# Autodesk Inventor assembly: zlozenie
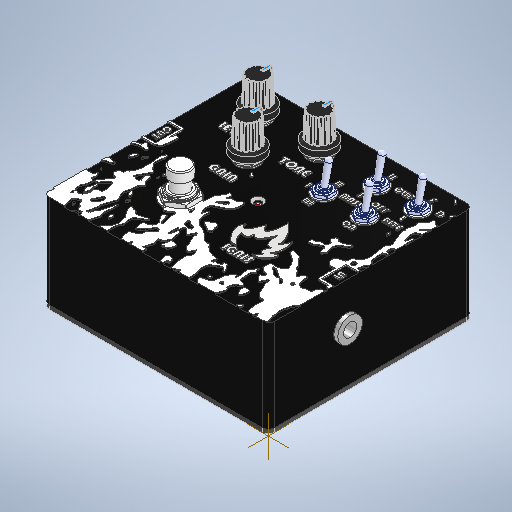
[picture p0: Inventor's stored thumbnail of the model, 512x512]
Saved by Autodesk Inventor 2025 (Build 290162000, 162)
## iProperties
Created: 2026-04-02
Part Number: zlozenie
Document SubType Name: Assembly
Designer: zzapa
Author: zzapa
## Documents named in this file (18)
- C:\Users\zzapa\Desktop\Projekty\elektronika\Ignis-overdrive\model\assembly.iam
- C:\Users\zzapa\Desktop\Projekty\elektronika\Ignis-overdrive\model\base.ipt
- C:\Users\zzapa\Desktop\Projekty\elektronika\Ignis-overdrive\model\enclosure.ipt
- C:\Users\zzapa\Documents\Inventor\Content Center Files\R2025\pl-PL\GB 809-88 B\Nut GB 809 B M2,5 x 6.ipt
- C:\Users\zzapa\Desktop\Projekty\elektronika\Ignis-overdrive\model\PotentiometerB10K.ipt
- C:\Users\zzapa\Desktop\Projekty\elektronika\Ignis-overdrive\model\knob.ipt
- C:\Users\zzapa\Desktop\Projekty\elektronika\Ignis-overdrive\model\Jack_enclosure.ipt
- C:\Users\zzapa\Desktop\Projekty\elektronika\Ignis-overdrive\model\Jack_inner.ipt
- C:\Users\zzapa\Desktop\Projekty\elektronika\Ignis-overdrive\model\9V_battery.ipt
- C:\Users\zzapa\Desktop\Projekty\elektronika\Ignis-overdrive\model\9V_input.ipt
- C:\Users\zzapa\Desktop\Projekty\elektronika\Ignis-overdrive\model\import\MTS-1xx-A1-blue\MTS-1xx-A1-blue-no-nuts.iam
- C:\Users\zzapa\Desktop\Projekty\elektronika\Ignis-overdrive\model\import\PCB_V1\PCB_V1.iam
- C:\Users\zzapa\Desktop\Projekty\elektronika\Ignis-overdrive\model\import\GŘRVA_MECHANO_3PDT_FOOTSWITCH\GŘRVA_MECHANO_3PDT_FOOTSWITCH.ipt
- C:\Users\zzapa\Desktop\Projekty\elektronika\Ignis-overdrive\model\import\M7 × 0.75 NUT\M7 × 0.75 NUT.ipt
- C:\Users\zzapa\Desktop\Projekty\elektronika\Ignis-overdrive\model\import\M12 NUT FOR FOOTSWITCH\M12 NUT FOR FOOTSWITCH.ipt
- C:\Users\zzapa\Desktop\Projekty\elektronika\Ignis-overdrive\model\import\MTS-1xx-A1-blue\MTS-1xx-NUT.ipt
- C:\Users\zzapa\Desktop\Projekty\elektronika\Ignis-overdrive\model\import\red-led-5mm\red-led-5mm.ipt
- C:\Users\zzapa\Desktop\Projekty\elektronika\Ignis-overdrive\model\led_holder.ipt
## Components (40 placed, 17 different names)
1. base:1 — Zestawiające:1, Zestawiające:2, Zestawiające:3, Zestawiające:4, Zestawiające:9, Zestawiające:87, Równoległe:19, Zestawiające:88
2. enclosure:1 — Zestawiające:3, Zestawiające:4, Zestawiające:5, Równoległe:1, Zestawiające:6, Równoległe:2, Zestawiające:7, Równoległe:3, Zestawiające:8, Równoległe:4, Zestawiające:9, Zestawiające:23, Zestawiające:24, Zestawiające:25, Zestawiające:26, Zestawiające:27, Zestawiające:28, Zestawiające:29, Równoległe:5, Zestawiające:32, Zestawiające:33, Zestawiające:47, Zestawiające:48, Zestawiające:49, Zestawiające:50, Zestawiające:51, Zestawiające:52, Zestawiające:53, Równoległe:10, Równoległe:11, Równoległe:12, Równoległe:13, Zestawiające:63, Zestawiające:64, Zestawiające:65, Zestawiające:66, Zestawiające:67, Zestawiające:68, Zestawiające:72, Zestawiające:74, Zestawiające:75, Zestawiające:76, Zestawiające:77, Zestawiające:78, Zestawiające:83, Zestawiające:84, Zestawiające:85, Zestawiające:86, Kątowe:43, Zestawiające:89, Zestawiające:90, Zestawiające:93, Zestawiające:94, Zestawiające:95, Równoległe:20, Równoległe:21
3. Nut GB/T 809-1988 Type B M2,5x6:1 — Zestawiające:5, Równoległe:1, Kątowe:1
4. Nut GB/T 809-1988 Type B M2,5x6:2 — Zestawiające:6, Równoległe:2, Kątowe:2
5. Nut GB/T 809-1988 Type B M2,5x6:3 — Zestawiające:7, Równoległe:3, Kątowe:3
6. Nut GB/T 809-1988 Type B M2,5x6:4 — Zestawiające:8, Równoległe:4, Kątowe:4
7. PotentiometerB10K:1 — Kątowe:5, Zestawiające:18, Zestawiające:19, Zestawiające:54
8. PotentiometerB10K:2 — Kątowe:6, Zestawiające:17, Zestawiające:20, Zestawiające:57
9. PotentiometerB10K:3 — Kątowe:7, Zestawiające:16, Zestawiające:21, Zestawiające:56
10. knob:1 — Zestawiające:17, Zestawiające:20, Kątowe:12, Zestawiające:71
11. knob:2 — Zestawiające:16, Zestawiające:21, Kątowe:13, Zestawiające:70
12. knob:3 — Zestawiające:18, Zestawiające:19, Kątowe:14, Zestawiające:69
13. Jack_enclosure:1 — Zestawiające:22, Zestawiające:25, Kątowe:11
14. Jack_inner:1 — Zestawiające:22, Zestawiające:23, Zestawiające:24, Kątowe:10
15. Jack_enclosure:2 — Zestawiające:26, Zestawiające:27, Kątowe:9
16. Jack_inner:2 — Zestawiające:28, Zestawiające:29, Kątowe:8
17. 9V_battery:1 — Kątowe:43, Zestawiające:87, Równoległe:19, Zestawiające:88
18. 9V_input:1 — Równoległe:5, Zestawiające:32, Zestawiające:33
19. PCB_V1:1 [sub-assembly] — Zestawiające:47, Zestawiające:48, Zestawiające:49
20. GŘRVA_MECHANO_3PDT_FOOTSWITCH:1 — Zestawiające:72, Zestawiające:73, Równoległe:14, Kątowe:34
21. Nut GB/T 809-1988 Type B M2,5x6:5 — Zestawiające:50, Równoległe:12, Kątowe:26
22. Nut GB/T 809-1988 Type B M2,5x6:6 — Zestawiające:52, Równoległe:11, Kątowe:27
23. Nut GB/T 809-1988 Type B M2,5x6:7 — Zestawiające:53, Równoległe:10, Kątowe:28
24. Nut GB/T 809-1988 Type B M2,5x6:8 — Zestawiające:51, Równoległe:13, Kątowe:29
25. M7 × 0.75 NUT:1 — Zestawiające:54, Kątowe:30, Zestawiające:66, Zestawiające:67, Zestawiające:69
26. M7 × 0.75 NUT:2 — Zestawiające:56, Kątowe:31, Zestawiające:63, Zestawiające:68, Zestawiające:70
27. M7 × 0.75 NUT:3 — Kątowe:32, Zestawiające:57, Zestawiające:64, Zestawiające:65, Zestawiające:71
28. M12 NUT FOR FOOTSWITCH:1 — Kątowe:33, Zestawiające:73, Równoległe:14, Zestawiające:74
29. MTS-1xx-A1-blue-no-nuts:1 [sub-assembly] — Zestawiające:75, Zestawiające:80, Równoległe:16, Kątowe:39
30. MTS-1xx-A1-blue-no-nuts:2 [sub-assembly] — Zestawiające:76, Zestawiające:81, Równoległe:18, Kątowe:40
31. MTS-1xx-A1-blue-no-nuts:3 [sub-assembly] — Zestawiające:77, Zestawiające:79, Równoległe:15, Kątowe:41
32. MTS-1xx-A1-blue-no-nuts:4 [sub-assembly] — Zestawiające:78, Zestawiające:82, Równoległe:17, Kątowe:42
33. MTS-1xx-NUT:1 — Zestawiające:82, Kątowe:35, Zestawiające:84, Równoległe:17
34. MTS-1xx-NUT:2 — Zestawiające:81, Kątowe:36, Zestawiające:83, Równoległe:18
35. MTS-1xx-NUT:3 — Zestawiające:80, Kątowe:37, Zestawiające:85, Równoległe:16
36. MTS-1xx-NUT:4 — Zestawiające:79, Kątowe:38, Zestawiające:86, Równoległe:15
37. red-led-5mm:1 — Zestawiające:91, Zestawiające:92, Zestawiające:93
38. led_holder:1 — Zestawiające:89, Zestawiające:90, Zestawiające:91, Zestawiające:92
39. Nut GB/T 809-1988 Type B M2,5x6:9 — Zestawiające:95, Równoległe:21
40. Nut GB/T 809-1988 Type B M2,5x6:10 — Zestawiające:94, Równoległe:20
## Relationships (117: Mate 68, Angle 32, Flush 17)
- Zestawiające:1 [Mate]: base:1
- Zestawiające:2 [Mate]: base:1
- Zestawiające:3 [Mate]: base:1 ↔ enclosure:1
- Zestawiające:4 [Mate]: base:1 ↔ enclosure:1
- Zestawiające:5 [Mate]: enclosure:1 ↔ Nut GB/T 809-1988 Type B M2,5x6:1
- Równoległe:1 [Flush]: enclosure:1 ↔ Nut GB/T 809-1988 Type B M2,5x6:1
- Zestawiające:6 [Mate]: enclosure:1 ↔ Nut GB/T 809-1988 Type B M2,5x6:2
- Równoległe:2 [Flush]: enclosure:1 ↔ Nut GB/T 809-1988 Type B M2,5x6:2
- Zestawiające:7 [Mate]: enclosure:1 ↔ Nut GB/T 809-1988 Type B M2,5x6:3
- Równoległe:3 [Flush]: enclosure:1 ↔ Nut GB/T 809-1988 Type B M2,5x6:3
- Zestawiające:8 [Mate]: enclosure:1 ↔ Nut GB/T 809-1988 Type B M2,5x6:4
- Równoległe:4 [Flush]: enclosure:1 ↔ Nut GB/T 809-1988 Type B M2,5x6:4
- Kątowe:1 [Angle] (0 deg): Nut GB/T 809-1988 Type B M2,5x6:1
- Kątowe:2 [Angle] (0 deg): Nut GB/T 809-1988 Type B M2,5x6:2
- Kątowe:3 [Angle] (0 deg): Nut GB/T 809-1988 Type B M2,5x6:3
- Kątowe:4 [Angle] (0 deg): Nut GB/T 809-1988 Type B M2,5x6:4
- Zestawiające:9 [Mate]: base:1 ↔ enclosure:1
- Kątowe:5 [Angle] (0 deg): PotentiometerB10K:1
- Kątowe:6 [Angle] (0 deg): PotentiometerB10K:2
- Kątowe:7 [Angle] (0 deg): PotentiometerB10K:3
- Zestawiające:16 [Mate]: PotentiometerB10K:3 ↔ knob:2
- Zestawiające:17 [Mate]: PotentiometerB10K:2 ↔ knob:1
- Zestawiające:18 [Mate]: PotentiometerB10K:1 ↔ knob:3
- Zestawiające:19 [Mate]: PotentiometerB10K:1 ↔ knob:3
- Zestawiające:20 [Mate]: PotentiometerB10K:2 ↔ knob:1
- Zestawiające:21 [Mate]: PotentiometerB10K:3 ↔ knob:2
- Zestawiające:22 [Mate]: Jack_enclosure:1 ↔ Jack_inner:1
- Zestawiające:23 [Mate]: enclosure:1 ↔ Jack_inner:1
- Zestawiające:24 [Mate]: enclosure:1 ↔ Jack_inner:1
- Zestawiające:25 [Mate]: enclosure:1 ↔ Jack_enclosure:1
- Zestawiające:26 [Mate]: enclosure:1 ↔ Jack_enclosure:2
- Zestawiające:27 [Mate]: enclosure:1 ↔ Jack_enclosure:2
- Zestawiające:28 [Mate]: enclosure:1 ↔ Jack_inner:2
- Zestawiające:29 [Mate]: enclosure:1 ↔ Jack_inner:2
- Kątowe:8 [Angle] (0 deg): Jack_inner:2
- Kątowe:9 [Angle] (0 deg): Jack_enclosure:2
- Kątowe:10 [Angle] (0 deg): Jack_inner:1
- Kątowe:11 [Angle] (0 deg): Jack_enclosure:1
- Równoległe:5 [Flush]: enclosure:1 ↔ 9V_input:1
- Zestawiające:32 [Mate]: enclosure:1 ↔ 9V_input:1
- Zestawiające:33 [Mate]: enclosure:1 ↔ 9V_input:1
- Kątowe:12 [Angle] (180 deg): knob:1
- Kątowe:13 [Angle] (180 deg): knob:2
- Kątowe:14 [Angle] (180 deg): knob:3
- Zestawiające:47 [Mate]: enclosure:1 ↔ PCB_V1:1
- Zestawiające:48 [Mate]: enclosure:1 ↔ PCB_V1:1
- Zestawiające:49 [Mate]: enclosure:1 ↔ PCB_V1:1
- Zestawiające:50 [Mate]: enclosure:1 ↔ Nut GB/T 809-1988 Type B M2,5x6:5
- Zestawiające:51 [Mate]: enclosure:1 ↔ Nut GB/T 809-1988 Type B M2,5x6:8
- Zestawiające:52 [Mate]: enclosure:1 ↔ Nut GB/T 809-1988 Type B M2,5x6:6
- Zestawiające:53 [Mate]: enclosure:1 ↔ Nut GB/T 809-1988 Type B M2,5x6:7
- Równoległe:10 [Flush]: enclosure:1 ↔ Nut GB/T 809-1988 Type B M2,5x6:7
- Równoległe:11 [Flush]: enclosure:1 ↔ Nut GB/T 809-1988 Type B M2,5x6:6
- Równoległe:12 [Flush]: enclosure:1 ↔ Nut GB/T 809-1988 Type B M2,5x6:5
- Równoległe:13 [Flush]: enclosure:1 ↔ Nut GB/T 809-1988 Type B M2,5x6:8
- Kątowe:26 [Angle] (0 deg): Nut GB/T 809-1988 Type B M2,5x6:5
- Kątowe:27 [Angle] (0 deg): Nut GB/T 809-1988 Type B M2,5x6:6
- Kątowe:28 [Angle] (0 deg): Nut GB/T 809-1988 Type B M2,5x6:7
- Kątowe:29 [Angle] (0 deg): Nut GB/T 809-1988 Type B M2,5x6:8
- Zestawiające:54 [Mate]: PotentiometerB10K:1 ↔ M7 × 0.75 NUT:1
- Zestawiające:56 [Mate]: PotentiometerB10K:3 ↔ M7 × 0.75 NUT:2
- Kątowe:30 [Angle] (0 deg): M7 × 0.75 NUT:1
- Kątowe:31 [Angle] (0 deg): M7 × 0.75 NUT:2
- Kątowe:32 [Angle] (0 deg): M7 × 0.75 NUT:3
- Zestawiające:57 [Mate]: PotentiometerB10K:2 ↔ M7 × 0.75 NUT:3
- Kątowe:33 [Angle] (0 deg): M12 NUT FOR FOOTSWITCH:1
- Zestawiające:63 [Mate]: enclosure:1 ↔ M7 × 0.75 NUT:2
- Zestawiające:64 [Mate]: enclosure:1 ↔ M7 × 0.75 NUT:3
- Zestawiające:65 [Mate]: enclosure:1 ↔ M7 × 0.75 NUT:3
- Zestawiające:66 [Mate]: enclosure:1 ↔ M7 × 0.75 NUT:1
- Zestawiające:67 [Mate]: enclosure:1 ↔ M7 × 0.75 NUT:1
- Zestawiające:68 [Mate]: enclosure:1 ↔ M7 × 0.75 NUT:2
- Zestawiające:69 [Mate] (1 mm): knob:3 ↔ M7 × 0.75 NUT:1
- Zestawiające:70 [Mate] (1 mm): knob:2 ↔ M7 × 0.75 NUT:2
- Zestawiające:71 [Mate] (1 mm): knob:1 ↔ M7 × 0.75 NUT:3
- Zestawiające:72 [Mate]: enclosure:1 ↔ GŘRVA_MECHANO_3PDT_FOOTSWITCH:1
- Zestawiające:73 [Mate]: GŘRVA_MECHANO_3PDT_FOOTSWITCH:1 ↔ M12 NUT FOR FOOTSWITCH:1
- Równoległe:14 [Flush] (1.5 mm): GŘRVA_MECHANO_3PDT_FOOTSWITCH:1 ↔ M12 NUT FOR FOOTSWITCH:1
- Zestawiające:74 [Mate]: enclosure:1 ↔ M12 NUT FOR FOOTSWITCH:1
- Kątowe:34 [Angle] (0 deg): GŘRVA_MECHANO_3PDT_FOOTSWITCH:1
- Zestawiające:75 [Mate]: enclosure:1 ↔ MTS-1xx-A1-blue-no-nuts:1
- Zestawiające:76 [Mate]: enclosure:1 ↔ MTS-1xx-A1-blue-no-nuts:2
- Zestawiające:77 [Mate]: enclosure:1 ↔ MTS-1xx-A1-blue-no-nuts:3
- Zestawiające:78 [Mate]: enclosure:1 ↔ MTS-1xx-A1-blue-no-nuts:4
- Zestawiające:79 [Mate]: MTS-1xx-A1-blue-no-nuts:3 ↔ MTS-1xx-NUT:4
- Zestawiające:80 [Mate]: MTS-1xx-A1-blue-no-nuts:1 ↔ MTS-1xx-NUT:3
- Zestawiające:81 [Mate]: MTS-1xx-A1-blue-no-nuts:2 ↔ MTS-1xx-NUT:2
- Zestawiające:82 [Mate]: MTS-1xx-A1-blue-no-nuts:4 ↔ MTS-1xx-NUT:1
- Kątowe:35 [Angle] (0 deg): MTS-1xx-NUT:1
- Kątowe:36 [Angle] (0 deg): MTS-1xx-NUT:2
- Kątowe:37 [Angle] (0 deg): MTS-1xx-NUT:3
- Kątowe:38 [Angle] (0 deg): MTS-1xx-NUT:4
- Zestawiające:83 [Mate]: enclosure:1 ↔ MTS-1xx-NUT:2
- Zestawiające:84 [Mate]: enclosure:1 ↔ MTS-1xx-NUT:1
- Zestawiające:85 [Mate]: enclosure:1 ↔ MTS-1xx-NUT:3
- Zestawiające:86 [Mate]: enclosure:1 ↔ MTS-1xx-NUT:4
- Równoległe:15 [Flush] (-1 mm): MTS-1xx-A1-blue-no-nuts:3 ↔ MTS-1xx-NUT:4
- Równoległe:16 [Flush] (-1 mm): MTS-1xx-A1-blue-no-nuts:1 ↔ MTS-1xx-NUT:3
- Równoległe:17 [Flush] (-1 mm): MTS-1xx-A1-blue-no-nuts:4 ↔ MTS-1xx-NUT:1
- Równoległe:18 [Flush] (-1 mm): MTS-1xx-A1-blue-no-nuts:2 ↔ MTS-1xx-NUT:2
- Kątowe:39 [Angle] (0 deg): MTS-1xx-A1-blue-no-nuts:1
- Kątowe:40 [Angle] (0 deg): MTS-1xx-A1-blue-no-nuts:2
- Kątowe:41 [Angle] (0 deg): MTS-1xx-A1-blue-no-nuts:3
- Kątowe:42 [Angle] (0 deg): MTS-1xx-A1-blue-no-nuts:4
- Kątowe:43 [Angle] (0 deg): enclosure:1 ↔ 9V_battery:1
- Zestawiające:87 [Mate]: base:1 ↔ 9V_battery:1
- Równoległe:19 [Flush]: base:1 ↔ 9V_battery:1
- Zestawiające:88 [Mate]: base:1 ↔ 9V_battery:1
- Zestawiające:89 [Mate]: enclosure:1 ↔ led_holder:1
- Zestawiające:90 [Mate]: enclosure:1 ↔ led_holder:1
- Zestawiające:91 [Mate]: red-led-5mm:1 ↔ led_holder:1
- Zestawiające:92 [Mate]: red-led-5mm:1 ↔ led_holder:1
- Zestawiające:93 [Mate]: enclosure:1 ↔ red-led-5mm:1
- Zestawiające:94 [Mate]: enclosure:1 ↔ Nut GB/T 809-1988 Type B M2,5x6:10
- Zestawiające:95 [Mate]: enclosure:1 ↔ Nut GB/T 809-1988 Type B M2,5x6:9
- Równoległe:20 [Flush]: enclosure:1 ↔ Nut GB/T 809-1988 Type B M2,5x6:10
- Równoległe:21 [Flush]: enclosure:1 ↔ Nut GB/T 809-1988 Type B M2,5x6:9
